# Autodesk Inventor assembly: stepper_42
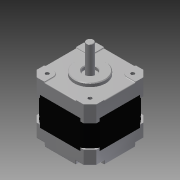
[picture p0: Inventor's stored thumbnail of the model, 180x180]
Saved by Autodesk Inventor 2013 (Build 170138000, 138)
## iProperties
Created: 2015-02-19
Part Number: stepper_42
Document SubType Name: Assembly
Designer: Noa Izumi
Author: Noa Izumi
## Documents named in this file (5)
- C:\reprap\TinyBoy_v3_20150220\stepper_42.iam
- C:\reprap\TinyBoy_v3_20150220\stepper_middle_42.ipt
- C:\reprap\TinyBoy_v3_20150220\stepper_bottom_42.ipt
- C:\reprap\TinyBoy_v3_20150220\stepper_front_42.ipt
- C:\reprap\TinyBoy_v3_20150220\screw_M3_5.ipt
## Components (7 placed, 4 different names)
1. stepper_middle_42:1 — 插入:1, 齊平:1, 插入:2, 齊平:2
2. stepper_bottom_42:1 — 插入:2, 齊平:2, 插入:3, 插入:4, 插入:5, 插入:6
3. stepper_front_42:1 — 插入:1, 齊平:1
4. screw_M3_5:1 — 插入:3
5. screw_M3_5:2 — 插入:5
6. screw_M3_5:3 — 插入:4
7. screw_M3_5:4 — 插入:6
## Relationships (8: Insert 6, Flush 2)
- 插入:1 [Insert]: stepper_middle_42:1 ↔ stepper_front_42:1
- 齊平:1 [Flush]: stepper_middle_42:1 ↔ stepper_front_42:1
- 插入:2 [Insert]: stepper_middle_42:1 ↔ stepper_bottom_42:1
- 齊平:2 [Flush]: stepper_middle_42:1 ↔ stepper_bottom_42:1
- 插入:3 [Insert]: stepper_bottom_42:1 ↔ screw_M3_5:1
- 插入:4 [Insert]: stepper_bottom_42:1 ↔ screw_M3_5:3
- 插入:5 [Insert]: stepper_bottom_42:1 ↔ screw_M3_5:2
- 插入:6 [Insert]: stepper_bottom_42:1 ↔ screw_M3_5:4
